# Autodesk Inventor assembly: bottom_board
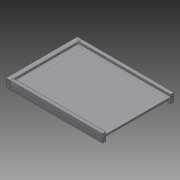
[picture p0: Inventor's stored thumbnail of the model, 180x180]
Saved by Autodesk Inventor 2014 SP1 (Build 180222100, 222)
## iProperties
Created: 2014-02-20
Part Number: bottom_board
Document SubType Name: Assembly
Designer: Chris
Mass: 3370.61 g
Surface Area: 6815.71 cm^2
Volume: 3370.61 cm^3
Density: 1 g/cm^3
Author: Chris
## Documents named in this file (4)
- C:\Users\Chris\Documents\projects\langstroth_plain\botton_board\bottom_board.iam
- C:\Users\Chris\Documents\projects\langstroth_plain\botton_board\bottom_board.ipt
- C:\Users\Chris\Documents\projects\langstroth_plain\botton_board\bottom_board_slat_back.ipt
- C:\Users\Chris\Documents\projects\langstroth_plain\botton_board\bottom_board_slat_side.ipt
## Components (4 placed, 3 different names)
1. bottom_board:1 — Mate:8, Mate:9, Mate:10, Mate:11, Flush:1, Mate:12, Mate:13, Mate:14, Flush:2
2. bottom_board_slat_back:1 — Mate:8, Mate:9, Mate:10
3. bottom_board_slat_side:1 — Mate:11, Flush:1, Mate:12
4. bottom_board_slat_side:2 — Mate:13, Mate:14, Flush:2
## Relationships (9: Mate 7, Flush 2)
- Mate:8: bottom_board:1 ↔ bottom_board_slat_back:1
- Mate:9: bottom_board:1 ↔ bottom_board_slat_back:1
- Mate:10: bottom_board:1 ↔ bottom_board_slat_back:1
- Mate:11: bottom_board:1 ↔ bottom_board_slat_side:1
- Flush:1: bottom_board:1 ↔ bottom_board_slat_side:1
- Mate:12: bottom_board:1 ↔ bottom_board_slat_side:1
- Mate:13: bottom_board:1 ↔ bottom_board_slat_side:2
- Mate:14: bottom_board:1 ↔ bottom_board_slat_side:2
- Flush:2: bottom_board:1 ↔ bottom_board_slat_side:2
